# Autodesk Inventor assembly: april_assembly
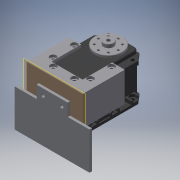
[picture p0: Inventor's stored thumbnail of the model, 180x180]
Saved by Autodesk Inventor 2018 (Build 220112000, 112)
## iProperties
Created: 2018-06-13
Part Number: april_assembly
Document SubType Name: Assembly
Designer: bitbots
Author: bitbots
## Documents named in this file (4)
- C:\Users\bitbots\Desktop\bitbots_hardware\davros\april_assembly.iam
- C:\minibot\motors\MX28\mx28_with_bearing.iam
- C:\Users\bitbots\Desktop\bitbots_hardware\davros\april_tag.ipt
- C:\Users\bitbots\Desktop\bitbots_hardware\davros\april_tag_2.ipt
## Components (3 placed, 3 different names)
1. mx28_with_bearing:1 [sub-assembly] — Flush:1, Flush:2
2. april_tag:1 — Flush:1, Flush:2, Flush:3, Flush:4
3. april_tag_2:1 — Flush:3, Flush:4
## Relationships (4: Flush 4)
- Flush:1: mx28_with_bearing:1 ↔ april_tag:1
- Flush:2: mx28_with_bearing:1 ↔ april_tag:1
- Flush:3: april_tag:1 ↔ april_tag_2:1
- Flush:4: april_tag:1 ↔ april_tag_2:1
